# Autodesk Inventor assembly: 脚一枚
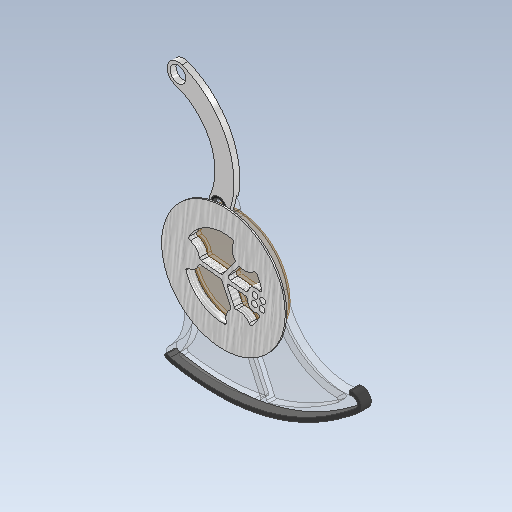
[picture p0: Inventor's stored thumbnail of the model, 512x512]
Saved by Autodesk Inventor 2020.2 (Build 242310000, 310)
## iProperties
Created: 2020-04-13
Part Number: 脚一枚
Document SubType Name: Assembly
Designer: aoyama
Mass: 30.4525 g
Surface Area: 259.988 cm^2
Volume: 17.8864 cm^3
Density: 1.70256 g/cm^3
Author: aoyama
## Documents named in this file (8)
- C:\Users\aoyam\Desktop\SRDC_local\Inventor\二年機\Geminiβ\脚\ネジクランク\脚一枚.iam
- C:\Users\aoyam\Desktop\SRDC_local\Inventor\二年機\Geminiβ\脚\ネジクランク\クランク3t.ipt
- C:\Users\aoyam\Desktop\SRDC_local\Inventor\二年機\Geminiβ\脚\ネジクランク\クランク4t.ipt
- C:\Users\aoyam\Desktop\SRDC_local\Inventor\二年機\Geminiβ\汎用部品\ベアリングd3D8B4F無.ipt
- C:\Users\aoyam\Desktop\SRDC_local\Inventor\二年機\Geminiβ\脚\ネジクランク\ヘッケン改.ipt
- C:\Users\aoyam\Desktop\SRDC_local\Inventor\二年機\Geminiβ\脚\ネジクランク\揺動節.ipt
- C:\Users\aoyam\Desktop\SRDC_local\Inventor\二年機\Geminiβ\汎用部品\オイレス外径8内径6L2.ipt
- C:\Users\aoyam\Desktop\SRDC_local\Inventor\二年機\Geminiβ\脚\ネジクランク\脚ゴム.ipt
## Components (9 placed, 7 different names)
1. クランク3t:1 — 挿入:15, 挿入:16, 挿入:17
2. クランク4t:1 — 挿入:12, 挿入:13, 挿入:14, 挿入:16
3. ベアリングd3D8B4F無:1 — 挿入:14
4. ベアリングd3D8B4F無:2 — 挿入:13, 挿入:15
5. ベアリングd3D8B4F無:3 — 挿入:12
6. ヘッケン改:1 — 挿入:8, 挿入:9, 挿入:11, 挿入:17, 挿入:18
7. 揺動節:1 — 挿入:11
8. オイレス外径8内径6L2:1 — 挿入:8
9. 脚ゴム:1 — 挿入:9, 挿入:18
## Relationships (10: Insert 10)
- 挿入:8 [Insert]: ヘッケン改:1 ↔ オイレス外径8内径6L2:1
- 挿入:9 [Insert]: ヘッケン改:1 ↔ 脚ゴム:1
- 挿入:11 [Insert]: ヘッケン改:1 ↔ 揺動節:1
- 挿入:12 [Insert]: クランク4t:1 ↔ ベアリングd3D8B4F無:3
- 挿入:13 [Insert]: クランク4t:1 ↔ ベアリングd3D8B4F無:2
- 挿入:14 [Insert]: クランク4t:1 ↔ ベアリングd3D8B4F無:1
- 挿入:15 [Insert]: クランク3t:1 ↔ ベアリングd3D8B4F無:2
- 挿入:16 [Insert]: クランク3t:1 ↔ クランク4t:1
- 挿入:17 [Insert] (0.2 mm): クランク3t:1 ↔ ヘッケン改:1
- 挿入:18 [Insert]: ヘッケン改:1 ↔ 脚ゴム:1
